# Autodesk Inventor assembly: Bouton poussoir NO
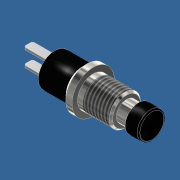
[picture p0: Inventor's stored thumbnail of the model, 180x180]
Saved by Autodesk Inventor 2015 SP2 (Build 190223200, 223)
## iProperties
Created: 2017-10-31
Part Number: Bouton poussoir NO
Project: Nom Projet
Description: Ens. Nom Ensemble
Document SubType Name: Assembly
Designer: Alexandre.PICOTTE
Author: Alexandre.PICOTTE
## Documents named in this file (3)
- P:\Electronique\Manette\Bouton poussoir NO.iam
- P:\Electronique\Manette\Bouton.ipt
- P:\Electronique\Manette\Capuchon.ipt
## Components (2 placed, 2 different names)
1. Bouton:1 — Logement:1
2. Capuchon:1 — Logement:1
## Relationships (1: Insert 1)
- Logement:1 [Insert]: Bouton:1 ↔ Capuchon:1
